# Autodesk Inventor assembly: Tamale Assembly Plate FLEX Assembly V1
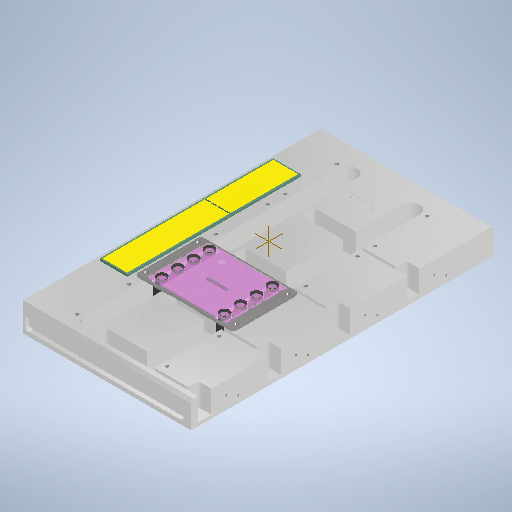
[picture p0: Inventor's stored thumbnail of the model, 512x512]
Saved by Autodesk Inventor 2025 (Build 290162000, 162)
## iProperties
Created: 2024-08-05
Part Number: Tamale Assembly Plate FLEX Assembly V1
Document SubType Name: Assembly
Designer: Caleb Fangmeier
Author: Caleb Fangmeier
## Documents named in this file (8)
- C:\Users\cfang\Desktop\nebraska-silicon-lab\Hardware\ETL\Module Assembly\Tamale Assembly Plate FLEX V1\Tamale Assembly Plate FLEX Assembly V1.iam
- C:\Users\cfang\Desktop\nebraska-silicon-lab\Hardware\ETL\Module Assembly\Tamale Assembly Plate FLEX V1\Tamale Assembly Plate FLEX V1.ipt
- C:\Users\cfang\Desktop\nebraska-silicon-lab\Hardware\ETL\Module Assembly\Tamale Assembly Plate FLEX V1\Flex Cable Assembly V1.iam
- C:\Users\cfang\Desktop\nebraska-silicon-lab\Hardware\ETL\Module Assembly\Tamale Assembly Plate FLEX V1\5427A604_Vacuum Cup.ipt
- C:\Users\cfang\Desktop\nebraska-silicon-lab\Hardware\ETL\Module Assembly\Tamale Assembly Plate FLEX V1\etl_etroc_module_v21\etl_etroc_module_v21.ipt
- C:\Users\cfang\Desktop\nebraska-silicon-lab\Hardware\ETL\Module Assembly\Tamale Assembly Plate FLEX V1\flex spacer V1.ipt
- C:\Users\cfang\Desktop\nebraska-silicon-lab\Hardware\ETL\Module Assembly\Tamale Assembly Plate FLEX V1\tamale_flex\tamale_flex.iam
- C:\Users\cfang\Desktop\nebraska-silicon-lab\Hardware\ETL\Module Assembly\Tamale Assembly Plate FLEX V1\wirebonder_coupon - V2\wirebonder_coupon - V2.iam
## Components (14 placed, 7 different names)
1. Tamale Assembly Plate FLEX V1:1 — Mate:1, Mate:2, Mate:4, Insert:4, Insert:5, Insert:6, Insert:7, Insert:8, Insert:9, Insert:10, Insert:11, Insert:12, Insert:13, Insert:14, Insert:15, Mate:6, Flush:3, Flush:4
2. Flex Cable Assembly V1:1 [sub-assembly] — Mate:1, Mate:2, Mate:4
3. etl_etroc_module_v21:1 — Mate:5, Flush:1, Flush:2
4. flex spacer V1:1 — Insert:12, Insert:13, Mate:5, Flush:1, Flush:2
5. 5427A604_Vacuum Cup:3 — Insert:4
6. 5427A604_Vacuum Cup:4 — Insert:6
7. 5427A604_Vacuum Cup:5 — Insert:7
8. 5427A604_Vacuum Cup:6 — Insert:11
9. 5427A604_Vacuum Cup:7 — Insert:5
10. 5427A604_Vacuum Cup:8 — Insert:8
11. 5427A604_Vacuum Cup:9 — Insert:9
12. 5427A604_Vacuum Cup:10 — Insert:10
13. tamale_flex:1 [sub-assembly] — Insert:14, Insert:15
14. wirebonder_coupon - V2:1 [sub-assembly] — Mate:6, Flush:3, Flush:4
## Relationships (21: Insert 12, Mate 5, Flush 4)
- Mate:1: Tamale Assembly Plate FLEX V1:1 ↔ Flex Cable Assembly V1:1
- Mate:2: Tamale Assembly Plate FLEX V1:1 ↔ Flex Cable Assembly V1:1
- Mate:4: Tamale Assembly Plate FLEX V1:1 ↔ Flex Cable Assembly V1:1
- Insert:4: Tamale Assembly Plate FLEX V1:1 ↔ 5427A604_Vacuum Cup:3
- Insert:5: Tamale Assembly Plate FLEX V1:1 ↔ 5427A604_Vacuum Cup:7
- Insert:6: Tamale Assembly Plate FLEX V1:1 ↔ 5427A604_Vacuum Cup:4
- Insert:7: Tamale Assembly Plate FLEX V1:1 ↔ 5427A604_Vacuum Cup:5
- Insert:8: Tamale Assembly Plate FLEX V1:1 ↔ 5427A604_Vacuum Cup:8
- Insert:9: Tamale Assembly Plate FLEX V1:1 ↔ 5427A604_Vacuum Cup:9
- Insert:10: Tamale Assembly Plate FLEX V1:1 ↔ 5427A604_Vacuum Cup:10
- Insert:11: Tamale Assembly Plate FLEX V1:1 ↔ 5427A604_Vacuum Cup:6
- Insert:12: Tamale Assembly Plate FLEX V1:1 ↔ flex spacer V1:1
- Insert:13: Tamale Assembly Plate FLEX V1:1 ↔ flex spacer V1:1
- Insert:14: Tamale Assembly Plate FLEX V1:1 ↔ tamale_flex:1
- Insert:15: Tamale Assembly Plate FLEX V1:1 ↔ tamale_flex:1
- Mate:5: etl_etroc_module_v21:1 ↔ flex spacer V1:1
- Flush:1 (1 mm): etl_etroc_module_v21:1 ↔ flex spacer V1:1
- Flush:2 (7 mm): etl_etroc_module_v21:1 ↔ flex spacer V1:1
- Mate:6: Tamale Assembly Plate FLEX V1:1 ↔ wirebonder_coupon - V2:1
- Flush:3 (5 mm): Tamale Assembly Plate FLEX V1:1 ↔ wirebonder_coupon - V2:1
- Flush:4 (40 mm): Tamale Assembly Plate FLEX V1:1 ↔ wirebonder_coupon - V2:1
